# Autodesk Inventor assembly: demo_1
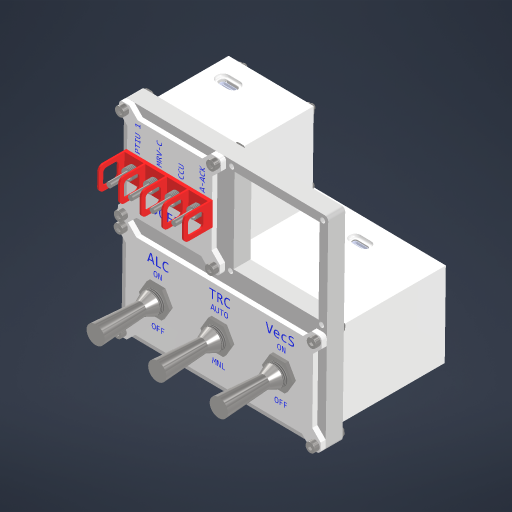
[picture p0: Inventor's stored thumbnail of the model, 512x512]
Saved by Autodesk Inventor 2024 (Build 280153000, 153)
## iProperties
Created: 2026-05-08
Part Number: demo_1
Document SubType Name: Assembly
Designer: schar
Author: schar
## Documents named in this file (7)
- C:\Users\schar\Desktop\MHIPS\models\racks\assembled\demo_1.iam
- C:\Users\schar\Desktop\MHIPS\models\tiles\2x1\lvl202x01_t\lvl202x01.iam
- C:\Users\schar\Desktop\MHIPS\models\tiles\1x1\lvl301x01_4t\1x1_asm_main.iam
- C:\Users\schar\Desktop\MHIPS\models\racks\frames\frame_demo_2x2_xyxx.ipt
- C:\Users\schar\Documents\Inventor\Content Center Files\R2024\en-US\AS 1420\AS 1420 - 1973 - M3 x 16.ipt
- C:\Users\schar\Documents\Inventor\Content Center Files\R2024\en-US\DIN 439-2\DIN 439 - M3 x 0,5.ipt
- C:\Users\schar\Documents\Inventor\Content Center Files\R2024\en-US\DIN 439-2\DIN 439 - M2,5 x 0,45.ipt
## Components (19 placed, 6 different names)
1. lvl202x01:1 [sub-assembly] — Mate:1, Flush:1, Flush:2, Insert:4, Insert:5, Insert:6, Insert:7
2. 1x1_asm_main:1 [sub-assembly] — Mate:1, Flush:1, Flush:2, Flush:3, Insert:2, Insert:3, Insert:8, Insert:9
3. frame_demo_2x2_xyxx:1 — Flush:3, Mate:3, Mate:5, Mate:7, Mate:9, Mate:11, Insert:10, Mate:13, Mate:15
4. AS 1420 - Metric M3 x 16:2 — Insert:2, Mate:4
5. AS 1420 - Metric M3 x 16:3 — Insert:3, Mate:8
6. AS 1420 - Metric M3 x 16:4 — Insert:4, Mate:10
7. AS 1420 - Metric M3 x 16:5 — Insert:5, Mate:14
8. AS 1420 - Metric M3 x 16:6 — Insert:6, Mate:12
9. AS 1420 - Metric M3 x 16:7 — Insert:7
10. AS 1420 - Metric M3 x 16:8 — Insert:8, Mate:6
11. AS 1420 - Metric M3 x 16:9 — Insert:9, Mate:2
12. DIN 439-2 - replaced by DIN EN 24035/28675 M3:1 — Mate:2, Mate:3
13. DIN 439-2 - replaced by DIN EN 24035/28675 M3:2 — Mate:4, Mate:5
14. DIN 439-2 - replaced by DIN EN 24035/28675 M3:3 — Mate:6, Mate:7
15. DIN 439-2 - replaced by DIN EN 24035/28675 M3:4 — Mate:8, Mate:9
16. DIN 439-2 - replaced by DIN EN 24035/28675 M3:5 — Mate:10, Mate:11
17. DIN 439-2 - replaced by DIN EN 24035/28675 M2,5:1 — Insert:10
18. DIN 439-2 - replaced by DIN EN 24035/28675 M3:6 — Mate:12, Mate:13
19. DIN 439-2 - replaced by DIN EN 24035/28675 M3:7 — Mate:14, Mate:15
## Relationships (27: Mate 15, Insert 9, Flush 3)
- Mate:1: lvl202x01:1 ↔ 1x1_asm_main:1
- Flush:1: lvl202x01:1 ↔ 1x1_asm_main:1
- Flush:2: lvl202x01:1 ↔ 1x1_asm_main:1
- Flush:3: 1x1_asm_main:1 ↔ frame_demo_2x2_xyxx:1
- Insert:2: 1x1_asm_main:1 ↔ AS 1420 - Metric M3 x 16:2
- Insert:3: 1x1_asm_main:1 ↔ AS 1420 - Metric M3 x 16:3
- Insert:4: lvl202x01:1 ↔ AS 1420 - Metric M3 x 16:4
- Insert:5: lvl202x01:1 ↔ AS 1420 - Metric M3 x 16:5
- Insert:6: lvl202x01:1 ↔ AS 1420 - Metric M3 x 16:6
- Insert:7: lvl202x01:1 ↔ AS 1420 - Metric M3 x 16:7
- Insert:8: 1x1_asm_main:1 ↔ AS 1420 - Metric M3 x 16:8
- Insert:9: 1x1_asm_main:1 ↔ AS 1420 - Metric M3 x 16:9
- Mate:2: AS 1420 - Metric M3 x 16:9 ↔ DIN 439-2 - replaced by DIN EN 24035/28675 M3:1
- Mate:3: frame_demo_2x2_xyxx:1 ↔ DIN 439-2 - replaced by DIN EN 24035/28675 M3:1
- Mate:4: AS 1420 - Metric M3 x 16:2 ↔ DIN 439-2 - replaced by DIN EN 24035/28675 M3:2
- Mate:5: frame_demo_2x2_xyxx:1 ↔ DIN 439-2 - replaced by DIN EN 24035/28675 M3:2
- Mate:6: AS 1420 - Metric M3 x 16:8 ↔ DIN 439-2 - replaced by DIN EN 24035/28675 M3:3
- Mate:7: frame_demo_2x2_xyxx:1 ↔ DIN 439-2 - replaced by DIN EN 24035/28675 M3:3
- Mate:8: AS 1420 - Metric M3 x 16:3 ↔ DIN 439-2 - replaced by DIN EN 24035/28675 M3:4
- Mate:9: frame_demo_2x2_xyxx:1 ↔ DIN 439-2 - replaced by DIN EN 24035/28675 M3:4
- Mate:10: AS 1420 - Metric M3 x 16:4 ↔ DIN 439-2 - replaced by DIN EN 24035/28675 M3:5
- Mate:11: frame_demo_2x2_xyxx:1 ↔ DIN 439-2 - replaced by DIN EN 24035/28675 M3:5
- Insert:10: frame_demo_2x2_xyxx:1 ↔ DIN 439-2 - replaced by DIN EN 24035/28675 M2,5:1
- Mate:12: AS 1420 - Metric M3 x 16:6 ↔ DIN 439-2 - replaced by DIN EN 24035/28675 M3:6
- Mate:13: frame_demo_2x2_xyxx:1 ↔ DIN 439-2 - replaced by DIN EN 24035/28675 M3:6
- Mate:14: AS 1420 - Metric M3 x 16:5 ↔ DIN 439-2 - replaced by DIN EN 24035/28675 M3:7
- Mate:15: frame_demo_2x2_xyxx:1 ↔ DIN 439-2 - replaced by DIN EN 24035/28675 M3:7
